# Autodesk Inventor assembly: 組合7
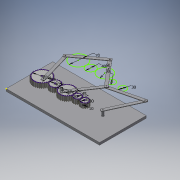
[picture p0: Inventor's stored thumbnail of the model, 180x180]
Saved by Autodesk Inventor 2019 (Build 230136000, 136)
## iProperties
Created: 2018-07-25
Part Number: 組合7
Material: 一般
Document SubType Name: Assembly
Designer: tronk
Author: tronk
## Documents named in this file (8)
- C:\Users\tronk\Desktop\tronk\0725\組合7.iam
- C:\Users\tronk\Desktop\tronk\零件8.ipt
- C:\Users\tronk\Desktop\tronk\0725\組合7\機械便覽魔法師\正齒輪1.iam
- C:\Users\tronk\Desktop\tronk\0725\組合7\機械便覽魔法師\正齒輪2.iam
- C:\Users\tronk\Desktop\tronk\0725\組合7\機械便覽魔法師\正齒輪3.iam
- C:\Users\tronk\Desktop\tronk\0725\組合7\機械便覽魔法師\正齒輪4.iam
- C:\Users\tronk\Desktop\tronk\0725\組合7\機械便覽魔法師\正齒輪5.iam
- C:\Users\tronk\Desktop\tronk\0725\零件15.ipt
## Components (12 placed, 3 different names)
1. 零件8:1 — 貼合:1, 貼合:2, 貼合:3, 貼合:4, 貼合:5, 齊平:1, 齊平:2, 齊平:3, 齊平:4, 齊平:5, 貼合:6, 貼合:7
2. 正齒輪:1 [sub-assembly] — 貼合:1, 齊平:1, 旋轉:1, 貼合:13
3. 正齒輪:2 [sub-assembly] — 貼合:2, 齊平:2, 旋轉:1, 旋轉:2
4. 正齒輪:3 [sub-assembly] — 貼合:3, 齊平:3, 旋轉:2, 旋轉:3, 貼合:11
5. 正齒輪:4 [sub-assembly] — 貼合:4, 齊平:4, 旋轉:3, 旋轉:4
6. 正齒輪:5 [sub-assembly] — 貼合:5, 齊平:5, 旋轉:4
7. 零件15:1 — 貼合:6, 貼合:7, 貼合:8, 貼合:9
8. 零件15:2 — 貼合:8, 貼合:9, 貼合:10, 貼合:12
9. 零件15:3 — 貼合:10, 貼合:11, 貼合:12, 貼合:14, 貼合:15
10. 零件15:4 — 貼合:13, 貼合:18, 貼合:19
11. 零件15:5 — 貼合:16, 貼合:17, 貼合:18, 貼合:19
12. 零件15:6 — 貼合:14, 貼合:15, 貼合:16, 貼合:17
## Relationships (28: Mate 19, Flush 5, RelateRotation 4)
- 貼合:1 [Mate]: 零件8:1 ↔ 正齒輪:1
- 貼合:2 [Mate]: 零件8:1 ↔ 正齒輪:2
- 貼合:3 [Mate]: 零件8:1 ↔ 正齒輪:3
- 貼合:4 [Mate]: 零件8:1 ↔ 正齒輪:4
- 貼合:5 [Mate]: 零件8:1 ↔ 正齒輪:5
- 齊平:1 [Flush]: 零件8:1 ↔ 正齒輪:1
- 齊平:2 [Flush]: 零件8:1 ↔ 正齒輪:2
- 齊平:3 [Flush]: 零件8:1 ↔ 正齒輪:3
- 齊平:4 [Flush]: 零件8:1 ↔ 正齒輪:4
- 齊平:5 [Flush]: 零件8:1 ↔ 正齒輪:5
- 旋轉:1 [RelateRotation] (1.857 ul): 正齒輪:1 ↔ 正齒輪:2
- 旋轉:2 [RelateRotation] (0.636 ul): 正齒輪:2 ↔ 正齒輪:3
- 旋轉:3 [RelateRotation] (2.2 ul): 正齒輪:3 ↔ 正齒輪:4
- 旋轉:4 [RelateRotation] (1 ul): 正齒輪:4 ↔ 正齒輪:5
- 貼合:6 [Mate]: 零件8:1 ↔ 零件15:1
- 貼合:7 [Mate]: 零件8:1 ↔ 零件15:1
- 貼合:8 [Mate]: 零件15:1 ↔ 零件15:2
- 貼合:9 [Mate]: 零件15:1 ↔ 零件15:2
- 貼合:10 [Mate]: 零件15:2 ↔ 零件15:3
- 貼合:11 [Mate]: 正齒輪:3 ↔ 零件15:3
- 貼合:12 [Mate]: 零件15:2 ↔ 零件15:3
- 貼合:13 [Mate]: 正齒輪:1 ↔ 零件15:4
- 貼合:14 [Mate]: 零件15:3 ↔ 零件15:6
- 貼合:15 [Mate]: 零件15:3 ↔ 零件15:6
- 貼合:16 [Mate]: 零件15:5 ↔ 零件15:6
- 貼合:17 [Mate]: 零件15:5 ↔ 零件15:6
- 貼合:18 [Mate]: 零件15:4 ↔ 零件15:5
- 貼合:19 [Mate]: 零件15:4 ↔ 零件15:5
